# Autodesk Inventor assembly: TestAssm
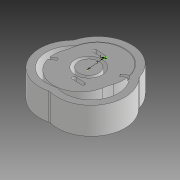
[picture p0: Inventor's stored thumbnail of the model, 180x180]
Saved by Autodesk Inventor 2020 (Build 240168000, 168)
## iProperties
Created: 2021-05-17
Part Number: TestAssm
Document SubType Name: Assembly
Designer: DDeGo
Author: DDeGo
## Documents named in this file (4)
- C:\Users\DDeGo\Documents\Drew\Projects\AirWankelEngine\cad\LiquidPiston V1\TestAssm.iam
- C:\Users\DDeGo\Documents\Drew\Projects\AirWankelEngine\cad\LiquidPiston V1\TestHousing.ipt
- C:\Users\DDeGo\Documents\Drew\Projects\AirWankelEngine\cad\LiquidPiston V1\TestRotor.ipt
- C:\Users\DDeGo\Documents\Drew\Projects\AirWankelEngine\cad\LiquidPiston V1\TestCam.ipt
## Components (3 placed, 3 different names)
1. TestHousing:1 — Mate:2, Mate:4
2. TestRotor:1 — Mate:2, Mate:3, Flush:1, Rotation:1
3. TestCam:1 — Mate:3, Mate:4, Flush:1, Rotation:1
## Relationships (5: Mate 3, Flush 1, RelateRotation 1)
- Mate:2: TestHousing:1 ↔ TestRotor:1
- Mate:3: TestRotor:1 ↔ TestCam:1
- Mate:4: TestHousing:1 ↔ TestCam:1
- Flush:1: TestRotor:1 ↔ TestCam:1
- Rotation:1 [RelateRotation] (2 ul): TestRotor:1 ↔ TestCam:1
